# Autodesk Inventor assembly: raspberry pi
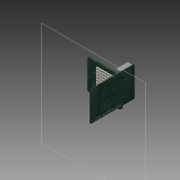
[picture p0: Inventor's stored thumbnail of the model, 180x180]
Saved by Autodesk Inventor 2015 (Build 190159000, 159)
## iProperties
Created: 2015-12-03
Part Number: raspberry pi
Document SubType Name: Assembly
Designer: david
Author: david
## Documents named in this file (6)
- Z:\gip\Inventor\generatie 7\Frame\Electronica\raspberry pi\raspberry pi.iam
- Z:\gip\Inventor\generatie 7\Frame\Electronica\raspberry pi\Bord.ipt
- Z:\gip\Inventor\generatie 7\Frame\Electronica\raspberry pi\USB.ipt
- Z:\gip\Inventor\generatie 7\Frame\Electronica\raspberry pi\gpio.iam
- Z:\gip\Inventor\generatie 7\Frame\Electronica\raspberry pi\netwerk.ipt
- Z:\gip\Inventor\generatie 7\Frame\Electronica\raspberry pi\hat.iam
## Components (6 placed, 5 different names)
1. Bord:1 — Mate:1, Mate:2, Flush:1, Flush:2, Flush:3, Mate:4, Flush:4, Flush:5, Mate:5, Flush:6, Mate:7, Angle:1
2. USB:1 — Mate:1, Flush:1, Mate:3, Flush:2
3. USB:2 — Mate:2, Mate:3, Flush:3, Mate:6
4. gpio:2 [sub-assembly] — Mate:4, Flush:4, Flush:5, Mate:8
5. netwerk:1 — Mate:5, Mate:6, Flush:6
6. hat:1 [sub-assembly] — Mate:7, Mate:8, Angle:1
## Relationships (15: Mate 8, Flush 6, Angle 1)
- Mate:1: Bord:1 ↔ USB:1
- Mate:2: Bord:1 ↔ USB:2
- Flush:1 (5 mm): Bord:1 ↔ USB:1
- Mate:3 (4 mm): USB:1 ↔ USB:2
- Flush:2: Bord:1 ↔ USB:1
- Flush:3: Bord:1 ↔ USB:2
- Mate:4: Bord:1 ↔ gpio:2
- Flush:4 (-1 mm): Bord:1 ↔ gpio:2
- Flush:5 (8 mm): Bord:1 ↔ gpio:2
- Mate:5: Bord:1 ↔ netwerk:1
- Mate:6 (2 mm): USB:2 ↔ netwerk:1
- Flush:6 (-1 mm): Bord:1 ↔ netwerk:1
- Mate:7: Bord:1 ↔ hat:1
- Mate:8: gpio:2 ↔ hat:1
- Angle:1 (0 deg): Bord:1 ↔ hat:1
